# Autodesk Inventor assembly: Glyph Lift System
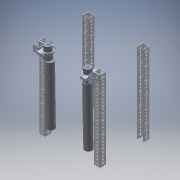
[picture p0: Inventor's stored thumbnail of the model, 180x180]
Saved by Autodesk Inventor 2017 (Build 210142000, 142)
## iProperties
Created: 2017-09-30
Part Number: Glyph Lift System
Document SubType Name: Assembly
Designer: Kenneth
Author: Kenneth
## Documents named in this file (6)
- C:\Workspaces\CAD\Glyph Lift System.iam
- C:\Workspaces\CAD\Spectrum-CAD-Library\FTC\FTC Tetrix KOP\Channel 416mm.ipt
- C:\Workspaces\CAD\Spectrum-CAD-Library\FTC\FTC Tetrix KOP\DC Motor Mount.ipt
- C:\Workspaces\CAD\Spectrum-CAD-Library\FTC\FTC Tetrix KOP\DC Gearhead Motor.ipt
- C:\Workspaces\CAD\Spectrum-CAD-Library\FTC\FTC Tetrix KOP\Channel 32mm.ipt
- C:\Workspaces\CAD\Intake roller.ipt
## Components (12 placed, 5 different names)
1. Channel 416mm:1 — Mate:3, Flush:1, Mate:4, Mate:5, Flush:3, Mate:11, Mate:12, Flush:5
2. Channel 416mm:2 — Mate:1, Mate:2, Flush:2, Flush:6
3. Channel 416mm:3 — Mate:3, Flush:2, Mate:6, Mate:7, Flush:4, Mate:8, Mate:9, Flush:5, Flush:6
4. Channel 416mm:4 — Mate:1, Mate:2, Flush:1
5. DC Motor Mount:1 — Mate:11, Mate:12, Mate:13, Mate:15, Mate:21
6. DC Motor Mount:2 — Mate:8, Mate:9, Mate:10, Mate:14, Mate:20
7. DC Gearhead Motor:1 — Mate:15, Mate:16, Mate:19, Mate:21
8. DC Gearhead Motor:2 — Mate:14, Mate:17, Mate:18, Mate:20
9. Channel 32mm:1 — Mate:4, Mate:5, Flush:3, Mate:13
10. Channel 32mm:2 — Mate:6, Mate:7, Flush:4, Mate:10
11. Intake roller:1 — Mate:16, Mate:19
12. Intake roller:2 — Mate:17, Mate:18
## Relationships (27: Mate 21, Flush 6)
- Mate:1: Channel 416mm:2 ↔ Channel 416mm:4
- Mate:2: Channel 416mm:2 ↔ Channel 416mm:4
- Mate:3: Channel 416mm:1 ↔ Channel 416mm:3
- Flush:1: Channel 416mm:1 ↔ Channel 416mm:4
- Flush:2: Channel 416mm:2 ↔ Channel 416mm:3
- Mate:4: Channel 416mm:1 ↔ Channel 32mm:1
- Mate:5: Channel 416mm:1 ↔ Channel 32mm:1
- Flush:3: Channel 416mm:1 ↔ Channel 32mm:1
- Mate:6: Channel 416mm:3 ↔ Channel 32mm:2
- Mate:7: Channel 416mm:3 ↔ Channel 32mm:2
- Flush:4: Channel 416mm:3 ↔ Channel 32mm:2
- Mate:8: Channel 416mm:3 ↔ DC Motor Mount:2
- Mate:9: Channel 416mm:3 ↔ DC Motor Mount:2
- Mate:10: DC Motor Mount:2 ↔ Channel 32mm:2
- Mate:11: Channel 416mm:1 ↔ DC Motor Mount:1
- Mate:12: Channel 416mm:1 ↔ DC Motor Mount:1
- Mate:13: DC Motor Mount:1 ↔ Channel 32mm:1
- Flush:5: Channel 416mm:1 ↔ Channel 416mm:3
- Mate:14: DC Motor Mount:2 ↔ DC Gearhead Motor:2
- Mate:15: DC Motor Mount:1 ↔ DC Gearhead Motor:1
- Flush:6: Channel 416mm:2 ↔ Channel 416mm:3
- Mate:16: DC Gearhead Motor:1 ↔ Intake roller:1
- Mate:17: DC Gearhead Motor:2 ↔ Intake roller:2
- Mate:18: DC Gearhead Motor:2 ↔ Intake roller:2
- Mate:19: DC Gearhead Motor:1 ↔ Intake roller:1
- Mate:20 (25.4 mm): DC Motor Mount:2 ↔ DC Gearhead Motor:2
- Mate:21 (25.4 mm): DC Motor Mount:1 ↔ DC Gearhead Motor:1
